# Autodesk Inventor assembly: EBoard
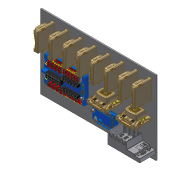
[picture p0: Inventor's stored thumbnail of the model, 180x180]
Saved by Autodesk Inventor 2012 (Build 160160000, 160)
## iProperties
Created: 2012-01-17
Part Number: EBoard
Document SubType Name: Assembly
Designer: JesseK
Author: JesseK
## Documents named in this file (6)
- Z:\UserData\Documents\Inventor\team1885frc\Robot2012\EBoard.iam
- Z:\UserData\Documents\Inventor\team1885frc\Robot2012\ElectronicsBoardConcept.ipt
- Z:\UserData\Documents\Inventor\team1885frc\Electronics\Jag\Jag.iam
- Z:\UserData\Documents\Inventor\team1885frc\Electronics\DigitalSidecar\elc_Digital_Sidecar_inv.iam
- Z:\UserData\Documents\Inventor\team1885frc\Electronics\PowerDistributionBoard\elc_Power_Distro_inv.iam
- Z:\UserData\Documents\Inventor\team1885frc\Electronics\cRIO_4Slot\Imported Components\cu_crio-9075_4-slot\cu_crio-9075_4-slot.ipt
## Components (14 placed, 5 different names)
1. ElectronicsBoardConcept:1 — Mate:20, Mate:21, Mate:22, Flush:14, Mate:23, Mate:24, Mate:25, Mate:26, Mate:27, Mate:28, Mate:29, Mate:30, Mate:31, Mate:32, Flush:23, Flush:24, Mate:40, Mate:41
2. elc_Digital_Sidecar_inv:1 [sub-assembly] — Mate:21, Flush:14
3. elc_Power_Distro_inv:1 [sub-assembly] — Mate:20, Flush:24
4. cu_crio-9075_4-slot:1 — Mate:22
5. Jag:1 [sub-assembly] — Mate:24, Flush:20, Flush:21, Mate:37, Mate:38
6. Jag:2 [sub-assembly] — Mate:26, Flush:18, Flush:19, Mate:35, Mate:36
7. Jag:3 [sub-assembly] — Mate:28, Flush:16, Flush:17, Mate:33, Mate:34
8. Jag:4 [sub-assembly] — Mate:23, Flush:21, Flush:22, Mate:38, Mate:39
9. Jag:5 [sub-assembly] — Mate:25, Flush:19, Flush:20, Mate:36, Mate:37
10. Jag:6 [sub-assembly] — Mate:27, Flush:17, Flush:18, Mate:34, Mate:35
11. Jag:7 [sub-assembly] — Mate:29, Flush:16, Mate:33, Flush:23
12. Jag:8 [sub-assembly] — Mate:30, Flush:22, Mate:39
13. Jag:9 [sub-assembly] — Mate:31, Mate:40
14. Jag:10 [sub-assembly] — Mate:32, Mate:41
## Relationships (32: Mate 22, Flush 10)
- Mate:20: ElectronicsBoardConcept:1 ↔ elc_Power_Distro_inv:1
- Mate:21: ElectronicsBoardConcept:1 ↔ elc_Digital_Sidecar_inv:1
- Mate:22 (6.35 mm): ElectronicsBoardConcept:1 ↔ cu_crio-9075_4-slot:1
- Flush:14 (38.1 mm): ElectronicsBoardConcept:1 ↔ elc_Digital_Sidecar_inv:1
- Mate:23: ElectronicsBoardConcept:1 ↔ Jag:4
- Mate:24: ElectronicsBoardConcept:1 ↔ Jag:1
- Mate:25: ElectronicsBoardConcept:1 ↔ Jag:5
- Mate:26: ElectronicsBoardConcept:1 ↔ Jag:2
- Mate:27: ElectronicsBoardConcept:1 ↔ Jag:6
- Mate:28: ElectronicsBoardConcept:1 ↔ Jag:3
- Mate:29: ElectronicsBoardConcept:1 ↔ Jag:7
- Mate:30: ElectronicsBoardConcept:1 ↔ Jag:8
- Mate:31: ElectronicsBoardConcept:1 ↔ Jag:9
- Mate:32: ElectronicsBoardConcept:1 ↔ Jag:10
- Flush:16 (76.2 mm): Jag:3 ↔ Jag:7
- Flush:17 (76.2 mm): Jag:3 ↔ Jag:6
- Flush:18 (76.2 mm): Jag:2 ↔ Jag:6
- Flush:19 (76.2 mm): Jag:2 ↔ Jag:5
- Flush:20 (76.2 mm): Jag:1 ↔ Jag:5
- Flush:21 (76.2 mm): Jag:1 ↔ Jag:4
- Flush:22 (76.2 mm): Jag:4 ↔ Jag:8
- Mate:33: Jag:3 ↔ Jag:7
- Mate:34: Jag:3 ↔ Jag:6
- Mate:35: Jag:2 ↔ Jag:6
- Mate:36: Jag:2 ↔ Jag:5
- Mate:37: Jag:1 ↔ Jag:5
- Mate:38: Jag:1 ↔ Jag:4
- Mate:39: Jag:4 ↔ Jag:8
- Flush:23 (19.05 mm): ElectronicsBoardConcept:1 ↔ Jag:7
- Flush:24 (50.8 mm): ElectronicsBoardConcept:1 ↔ elc_Power_Distro_inv:1
- Mate:40 (-228.6 mm): ElectronicsBoardConcept:1 ↔ Jag:9
- Mate:41 (-228.6 mm): ElectronicsBoardConcept:1 ↔ Jag:10
